# Autodesk Inventor assembly: asmTemp
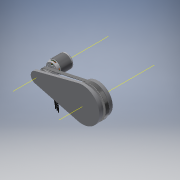
[picture p0: Inventor's stored thumbnail of the model, 180x180]
Saved by Autodesk Inventor 2018 (Build 220112000, 112)
## iProperties
Created: 2019-11-13
Part Number: asmTemp
Document SubType Name: Assembly
Designer: Bunny320
Author: Bunny320
## Documents named in this file (5)
- C:\Users\Bunny320\Desktop\sechs\4-CAD\asmTemp.iam
- C:\Users\Bunny320\Desktop\sechs\4-CAD\101-bottom.ipt
- C:\Users\Bunny320\Desktop\sechs\4-CAD\generated\J1_belt.iam
- C:\Users\Bunny320\Desktop\sechs\4-CAD\standardParts\61814-2RS1\61814-2RS1.iam
- C:\Users\Bunny320\Desktop\sechs\4-CAD\standardParts\turnigy sk3 4250 350kv\BLDC Motor Turnigy Aerodrive SK3 350KV Outrunner.iam
## Components (5 placed, 4 different names)
1. 101-bottom:1 — Flush:1, Flush:2, Flush:3
2. J1_belt:1 [sub-assembly] — Mate:1, Mate:2, Mate:3, Mate:4
3. 61814-2RS1:1 [sub-assembly] — Mate:2
4. 61814-2RS1:2 [sub-assembly] — Mate:3
5. BLDC Motor Turnigy Aerodrive SK3 350KV Outrunner:1 [sub-assembly] — Mate:4
## Relationships (7: Mate 4, Flush 3)
- Flush:1: 101-bottom:1
- Flush:2: 101-bottom:1
- Flush:3: 101-bottom:1
- Mate:1: J1_belt:1
- Mate:2: J1_belt:1 ↔ 61814-2RS1:1
- Mate:3: J1_belt:1 ↔ 61814-2RS1:2
- Mate:4: J1_belt:1 ↔ BLDC Motor Turnigy Aerodrive SK3 350KV Outrunner:1
